# Autodesk Inventor assembly: DoubleOdom
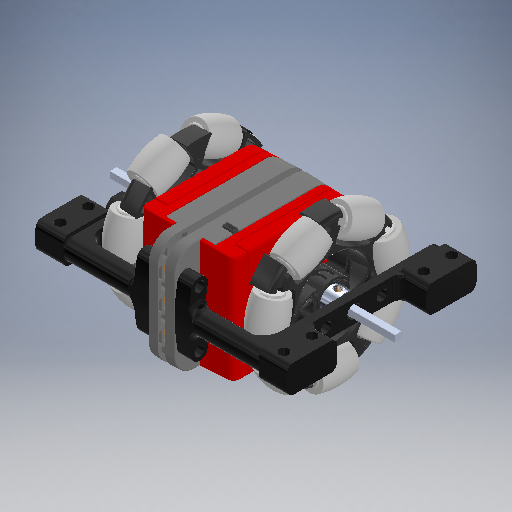
[picture p0: Inventor's stored thumbnail of the model, 512x512]
Saved by Autodesk Inventor 2026.1 (Build 301233000, 233)
## iProperties
Created: 2025-10-13
Part Number: DoubleOdom
Document SubType Name: Assembly
Designer: Teddy
Author: Teddy
## Documents named in this file (16)
- C:\Users\Teddy\Desktop\VexCAD\15InVEX\DoubleOdom.iam
- C:\Users\Teddy\Desktop\VexCAD\VEX-CAD-Inventor\Electronics\Sensors\Optical Shaft Encoder.ipt
- C:\Users\Teddy\Desktop\VexCAD\VEX-CAD-Inventor\Motion\Shaft LS\Shaft LS Capped\Shaft LS Capped 2.5.ipt
- C:\Users\Teddy\Desktop\VexCAD\VEX-CAD-Inventor\Motion\Shaft LS\Shaft LS Capped.ipt
- C:\Users\Teddy\Desktop\VexCAD\VEX-CAD-Inventor\Motion\Spacers\Spacer Nylon .375 OD.ipt
- C:\Users\Teddy\Desktop\VexCAD\VEX-CAD-Inventor\Motion\Spacers\Washer Teflon\TWasher .500 OD x .04000.ipt
- C:\Users\Teddy\Desktop\VexCAD\VEX-CAD-Inventor\Motion\Spacers\Washer Teflon.ipt
- C:\Users\Teddy\Desktop\VexCAD\VEX-CAD-Inventor\Motion\Shaft LS\Shaft Collar Metal\Shaft Collar No Screw.iam
- C:\Users\Teddy\Desktop\VexCAD\VEX-CAD-Inventor\Motion\Shaft LS\Shaft Collar Metal.iam
- C:\Users\Teddy\Desktop\VexCAD\VEX-CAD-Inventor\Motion\Wheels\Omni Wheel\2.75 Omni Half.ipt
- C:\Users\Teddy\Desktop\VexCAD\VEX-CAD-Inventor\Motion\Spacers\Spacer Nylon .375 OD\NSpacer .375 OD x .125.ipt
- C:\Users\Teddy\Desktop\VexCAD\15InVEX\DoublePod.ipt
- C:\Users\Teddy\Desktop\VexCAD\VEX-CAD-Inventor\Motion\Shaft LS\Bearing Flat.ipt
- C:\Users\Teddy\Desktop\VexCAD\VEX-CAD-Inventor\Structure\Hardware\Screw Steel - Star\SScrew Star Smooth .625.ipt
- C:\Users\Teddy\Desktop\VexCAD\VEX-CAD-Inventor\Structure\Hardware\Screw Steel - Star.ipt
- C:\Users\Teddy\Desktop\VexCAD\VEX-CAD-Inventor\Structure\Hardware\Nut Nylock.ipt
## Components (19 placed, 10 different names)
1. Optical Shaft Encoder:1 — Insert:1, Insert:3, Insert:9, Insert:10, Flush:2
2. Optical Shaft Encoder:2 — Insert:2, Insert:4, Insert:9, Insert:10, Insert:25, Insert:26
3. Shaft LS Capped 2.5:1 — Insert:1
4. Shaft LS Capped 2.5:2 — Insert:2
5. TWasher .500 OD x .04000:1 — Insert:3, Insert:19
6. TWasher .500 OD x .04000:2 — Insert:4, Insert:20
7. Shaft Collar No Screw:1 [sub-assembly] — Insert:18, Flush:1
8. Shaft Collar No Screw:2 [sub-assembly] — Insert:17, Insert:27
9. 2.75 Omni Half:1 — Insert:18, Insert:22
10. 2.75 Omni Half:2 — Insert:17, Insert:21
11. NSpacer .375 OD x .125:1 — Insert:19, Insert:22
12. NSpacer .375 OD x .125:2 — Insert:20, Insert:21
13. DoublePod:1 — Flush:1, Flush:2, Insert:23, Insert:24, Insert:30, Insert:31
14. Bearing Flat:1 — Insert:23, Insert:24, Insert:28, Insert:29
15. DoublePod:2 — Insert:25, Insert:26, Insert:27
16. SScrew Star Smooth .625:1 — Insert:28
17. SScrew Star Smooth .625:2 — Insert:29
18. Nut Nylock:1 — Insert:30
19. Nut Nylock:2 — Insert:31
## Relationships (23: Insert 21, Flush 2)
- Insert:1 (0.635 mm): Optical Shaft Encoder:1 ↔ Shaft LS Capped 2.5:1
- Insert:2 (0.635 mm): Optical Shaft Encoder:2 ↔ Shaft LS Capped 2.5:2
- Insert:3 (-1.397 mm): Optical Shaft Encoder:1 ↔ TWasher .500 OD x .04000:1
- Insert:4 (-1.397 mm): Optical Shaft Encoder:2 ↔ TWasher .500 OD x .04000:2
- Insert:9 (3.175 mm): Optical Shaft Encoder:1 ↔ Optical Shaft Encoder:2
- Insert:10 (3.175 mm): Optical Shaft Encoder:1 ↔ Optical Shaft Encoder:2
- Insert:17: Shaft Collar No Screw:2 ↔ 2.75 Omni Half:2
- Insert:18: Shaft Collar No Screw:1 ↔ 2.75 Omni Half:1
- Insert:19: TWasher .500 OD x .04000:1 ↔ NSpacer .375 OD x .125:1
- Insert:20: TWasher .500 OD x .04000:2 ↔ NSpacer .375 OD x .125:2
- Insert:21: 2.75 Omni Half:2 ↔ NSpacer .375 OD x .125:2
- Insert:22: 2.75 Omni Half:1 ↔ NSpacer .375 OD x .125:1
- Flush:1: Shaft Collar No Screw:1 ↔ DoublePod:1
- Flush:2: Optical Shaft Encoder:1 ↔ DoublePod:1
- Insert:23: DoublePod:1 ↔ Bearing Flat:1
- Insert:24: DoublePod:1 ↔ Bearing Flat:1
- Insert:25: Optical Shaft Encoder:2 ↔ DoublePod:2
- Insert:26: Optical Shaft Encoder:2 ↔ DoublePod:2
- Insert:27: Shaft Collar No Screw:2 ↔ DoublePod:2
- Insert:28: Bearing Flat:1 ↔ SScrew Star Smooth .625:1
- Insert:29: Bearing Flat:1 ↔ SScrew Star Smooth .625:2
- Insert:30: DoublePod:1 ↔ Nut Nylock:1
- Insert:31: DoublePod:1 ↔ Nut Nylock:2
